# Autodesk Inventor assembly: CycloidalGear
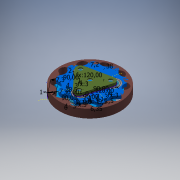
[picture p0: Inventor's stored thumbnail of the model, 180x180]
Saved by Autodesk Inventor 2018.3 (Build 223284000, 284)
## iProperties
Created: 2018-07-20
Part Number: CycloidalGear
Material: Generisch
Document SubType Name: Assembly
Designer: JochenAlt
Author: JochenAlt
## Documents named in this file (10)
- D:\Projects\FlowerPot\CAD\CycloidalGear\CycloidalGear.iam
- D:\Projects\FlowerPot\CAD\CycloidalGear\ExcentricShaft.ipt
- D:\Projects\FlowerPot\CAD\CycloidalGear\Excenter1.ipt
- D:\Projects\FlowerPot\CAD\CycloidalGear\Enclosure.ipt
- D:\Projects\FlowerPot\CAD\CycloidalGear\W 61701.iam
- D:\Projects\FlowerPot\CAD\CycloidalGear\Rotor.ipt
- D:\Projects\FlowerPot\CAD\CycloidalGear\Excenter2.ipt
- Excenter1.ipt
- D:\Projects\FlowerPot\CAD\CycloidalGear\ExcentricMotorShaft.ipt
- D:\Projects\FlowerPot\CAD\CycloidalGear\W 627_4-2Z.iam
## Components (20 placed, 7 different names)
1. Enclosure:1 — Passend:72, Passend:77, Fluchtend:24
2. W 61701:5 [sub-assembly] — Passend:15, Passend:26, Passend:29, Fluchtend:5, Passend:60, Fluchtend:10
3. ExcentricShaft:2 — Fluchtend:11, Passend:63, Fluchtend:12, Passend:80, Passend:87, Passend:89, Passend:93
4. ExcentricShaft:3 — Passend:15, Passend:26, Passend:29, Fluchtend:5, Fluchtend:23, Passend:83, Passend:86, Passend:91, Passend:94
5. ExcentricShaft:4 — Passend:57, Fluchtend:8, Fluchtend:21, Passend:82, Passend:84, Passend:92, Passend:95
6. Excenter1:2 — Passend:65, Fluchtend:15, Passend:70, Passend:76, Fluchtend:22, Fluchtend:23, Passend:81
7. W 61701:7 [sub-assembly] — Passend:63, Fluchtend:12, Passend:64, Fluchtend:13
8. W 61701:8 [sub-assembly] — Passend:57, Fluchtend:8, Passend:58, Fluchtend:14
9. W 61701:10 [sub-assembly] — Fluchtend:11, Passend:65, Passend:80
10. Rotor:1 — Passend:84, Passend:85, Passend:86, Passend:87, Passend:88
11. Excenter1:3 — Passend:58, Passend:60, Fluchtend:10, Passend:64, Fluchtend:13, Fluchtend:14, Passend:71, Fluchtend:18, Fluchtend:24, Drehung:1
12. MotorExcentricShaft:5 — Passend:68, Fluchtend:16, Passend:69, Passend:77, Fluchtend:22, Passend:78, Drehung:1, Passend:85, Passend:88, Passend:90, Passend:96
13. W 61701:11 [sub-assembly] — Fluchtend:15, Passend:81, Passend:83
14. W 61701:12 [sub-assembly] — Passend:68, Fluchtend:16, Passend:70
15. W 61701:13 [sub-assembly] — Passend:69, Passend:71, Fluchtend:18
16. W 61701:14 [sub-assembly] — Passend:76, Fluchtend:21, Passend:82
17. W 627_4-2Z:1 [sub-assembly] — Passend:89, Passend:93
18. W 627_4-2Z:2 [sub-assembly] — Passend:90, Passend:96
19. W 627_4-2Z:3 [sub-assembly] — Passend:92, Passend:95
20. W 627_4-2Z:4 [sub-assembly] — Passend:91, Passend:94
## Relationships (49: Mate 34, Flush 14, RelateRotation 1)
- Passend:15 [Mate]: W 61701:5 ↔ ExcentricShaft:3
- Passend:26 [Mate]: W 61701:5 ↔ ExcentricShaft:3
- Passend:29 [Mate]: W 61701:5 ↔ ExcentricShaft:3
- Fluchtend:5 [Flush]: W 61701:5 ↔ ExcentricShaft:3
- Passend:57 [Mate]: ExcentricShaft:4 ↔ W 61701:8
- Fluchtend:8 [Flush]: ExcentricShaft:4 ↔ W 61701:8
- Passend:58 [Mate]: W 61701:8 ↔ Excenter1:3
- Passend:60 [Mate]: W 61701:5 ↔ Excenter1:3
- Fluchtend:10 [Flush]: W 61701:5 ↔ Excenter1:3
- Fluchtend:11 [Flush]: ExcentricShaft:2 ↔ W 61701:10
- Passend:63 [Mate]: ExcentricShaft:2 ↔ W 61701:7
- Fluchtend:12 [Flush]: ExcentricShaft:2 ↔ W 61701:7
- Passend:64 [Mate]: W 61701:7 ↔ Excenter1:3
- Fluchtend:13 [Flush]: W 61701:7 ↔ Excenter1:3
- Passend:65 [Mate]: Excenter1:2 ↔ W 61701:10
- Fluchtend:14 [Flush]: W 61701:8 ↔ Excenter1:3
- Fluchtend:15 [Flush]: Excenter1:2 ↔ W 61701:11
- Passend:68 [Mate]: MotorExcentricShaft:5 ↔ W 61701:12
- Fluchtend:16 [Flush]: MotorExcentricShaft:5 ↔ W 61701:12
- Passend:69 [Mate]: MotorExcentricShaft:5 ↔ W 61701:13
- Passend:70 [Mate]: Excenter1:2 ↔ W 61701:12
- Passend:71 [Mate]: Excenter1:3 ↔ W 61701:13
- Fluchtend:18 [Flush]: Excenter1:3 ↔ W 61701:13
- Passend:72 [Mate]: Enclosure:1
- Passend:76 [Mate]: Excenter1:2 ↔ W 61701:14
- Fluchtend:21 [Flush]: ExcentricShaft:4 ↔ W 61701:14
- Passend:77 [Mate]: Enclosure:1 ↔ MotorExcentricShaft:5
- Fluchtend:22 [Flush]: Excenter1:2 ↔ MotorExcentricShaft:5
- Fluchtend:23 [Flush]: ExcentricShaft:3 ↔ Excenter1:2
- Fluchtend:24 [Flush]: Enclosure:1 ↔ Excenter1:3
- Passend:78 [Mate]: MotorExcentricShaft:5
- Drehung:1 [RelateRotation] (-0.1111 ul): Excenter1:3 ↔ MotorExcentricShaft:5
- Passend:80 [Mate]: ExcentricShaft:2 ↔ W 61701:10
- Passend:81 [Mate]: Excenter1:2 ↔ W 61701:11
- Passend:82 [Mate]: ExcentricShaft:4 ↔ W 61701:14
- Passend:83 [Mate]: ExcentricShaft:3 ↔ W 61701:11
- Passend:84 [Mate]: ExcentricShaft:4 ↔ Rotor:1
- Passend:85 [Mate]: Rotor:1 ↔ MotorExcentricShaft:5
- Passend:86 [Mate]: ExcentricShaft:3 ↔ Rotor:1
- Passend:87 [Mate]: ExcentricShaft:2 ↔ Rotor:1
- Passend:88 [Mate]: Rotor:1 ↔ MotorExcentricShaft:5
- Passend:89 [Mate]: ExcentricShaft:2 ↔ W 627_4-2Z:1
- Passend:90 [Mate]: MotorExcentricShaft:5 ↔ W 627_4-2Z:2
- Passend:91 [Mate]: ExcentricShaft:3 ↔ W 627_4-2Z:4
- Passend:92 [Mate]: ExcentricShaft:4 ↔ W 627_4-2Z:3
- Passend:93 [Mate]: ExcentricShaft:2 ↔ W 627_4-2Z:1
- Passend:94 [Mate]: ExcentricShaft:3 ↔ W 627_4-2Z:4
- Passend:95 [Mate]: ExcentricShaft:4 ↔ W 627_4-2Z:3
- Passend:96 [Mate]: MotorExcentricShaft:5 ↔ W 627_4-2Z:2
